# Autodesk Inventor assembly: tensegrity_revolute_joint_fixed
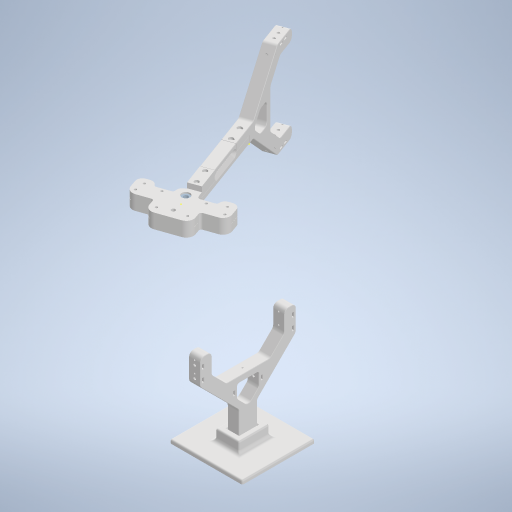
[picture p0: Inventor's stored thumbnail of the model, 512x512]
Saved by Autodesk Inventor 2023 (Build 270158000, 158)
## iProperties
Created: 2023-11-21
Part Number: tensegrity_revolute_joint_fixed
Document SubType Name: Assembly
Designer: zavrel
Author: zavrel
## Documents named in this file (9)
- C:\Users\zavrel\Documents\_OWNCLOUD_ACTUAL_WORK_AT_HOME\CLANEK_ustav\Tensegrity_Based_Joionts\03_winding_trajectory\models\tensegrity_revolute_joint_fixed.iam
- C:\Users\zavrel\Documents\_OWNCLOUD_ACTUAL_WORK_AT_HOME\CLANEK_ustav\Tensegrity_Based_Joionts\03_winding_trajectory\models\top.ipt
- C:\Users\zavrel\Documents\_OWNCLOUD_ACTUAL_WORK_AT_HOME\CLANEK_ustav\Tensegrity_Based_Joionts\03_winding_trajectory\models\bearing_d3D10b4.ipt
- C:\Users\zavrel\Documents\_OWNCLOUD_ACTUAL_WORK_AT_HOME\CLANEK_ustav\Tensegrity_Based_Joionts\03_winding_trajectory\models\bearing_d6D15b5.ipt
- C:\Users\zavrel\Documents\_OWNCLOUD_ACTUAL_WORK_AT_HOME\CLANEK_ustav\Tensegrity_Based_Joionts\03_winding_trajectory\models\middle_joint_v2.ipt
- C:\Users\zavrel\Documents\_OWNCLOUD_ACTUAL_WORK_AT_HOME\CLANEK_ustav\Tensegrity_Based_Joionts\03_winding_trajectory\models\middle_hole_v2.ipt
- C:\Users\zavrel\Documents\_OWNCLOUD_ACTUAL_WORK_AT_HOME\CLANEK_ustav\Tensegrity_Based_Joionts\03_winding_trajectory\models\middle_Y.ipt
- C:\Users\zavrel\Documents\_OWNCLOUD_ACTUAL_WORK_AT_HOME\CLANEK_ustav\Tensegrity_Based_Joionts\03_winding_trajectory\models\bottom.ipt
- C:\Users\zavrel\Documents\_OWNCLOUD_ACTUAL_WORK_AT_HOME\CLANEK_ustav\Tensegrity_Based_Joionts\03_winding_trajectory\models\base_frame.ipt
## Components (12 placed, 8 different names)
1. top:1 — Rotational:1, Rotational:2, Rotational:3, Rotational:4, Insert:2, Mate:2
2. bearing_d3D10b4:1 — Rotational:2
3. bearing_d3D10b4:2 — Rotational:1
4. bearing_d6D15b5:1 — Rotational:4, Rotational:5
5. bearing_d6D15b5:2 — Rotational:8
6. bearing_d6D15b5:3 — Rotational:3
7. middle_joint_v2:1 — Rotational:5, Insert:1, Mate:1
8. middle_hole_v2:1 — Rigid:1, Insert:1, Mate:1
9. middle_Y:1 — Rigid:1
10. top:2 — Rotational:8, Insert:2, Mate:2
11. bottom:1 — Rotational:7
12. base_frame:1 — Rotational:7
## Relationships (12: RevoluteJoint 7, Insert 2, Mate 2, WeldJoint 1)
- Rotational:1 [RevoluteJoint]: top:1 ↔ bearing_d3D10b4:2
- Rotational:2 [RevoluteJoint]: top:1 ↔ bearing_d3D10b4:1
- Rotational:3 [RevoluteJoint]: top:1 ↔ bearing_d6D15b5:3
- Rotational:4 [RevoluteJoint]: top:1 ↔ bearing_d6D15b5:1
- Rotational:5 [RevoluteJoint]: bearing_d6D15b5:1 ↔ middle_joint_v2:1
- Rigid:1 [WeldJoint]: middle_hole_v2:1 ↔ middle_Y:1
- Rotational:7 [RevoluteJoint]: bottom:1 ↔ base_frame:1
- Insert:1: middle_joint_v2:1 ↔ middle_hole_v2:1
- Mate:1: middle_joint_v2:1 ↔ middle_hole_v2:1
- Rotational:8 [RevoluteJoint]: bearing_d6D15b5:2 ↔ top:2
- Insert:2: top:1 ↔ top:2
- Mate:2: top:1 ↔ top:2
